# Autodesk Inventor assembly: Aspresor
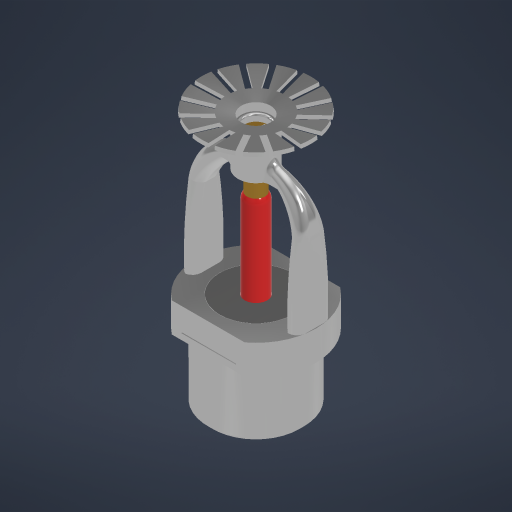
[picture p0: Inventor's stored thumbnail of the model, 512x512]
Saved by Autodesk Inventor 2024 (Build 280153000, 153)
## iProperties
Created: 2024-11-05
Part Number: Aspresor
Document SubType Name: Assembly
Designer: nesto
Author: nesto
## Documents named in this file (3)
- C:\Users\nesto\OneDrive - Universidad de la Sabana\Universidad\2024-2\CAD\Sistema de Riego\Aspresor.iam
- C:\Users\nesto\OneDrive - Universidad de la Sabana\Universidad\2024-2\CAD\Sistema de Riego\parte de abajo.ipt
- C:\Users\nesto\OneDrive - Universidad de la Sabana\Universidad\2024-2\CAD\Sistema de Riego\Parte de arriba aspresor.ipt
## Components (2 placed, 2 different names)
1. parte de abajo:1 — De rotación:1
2. Parte de arriba aspresor:1 — De rotación:1
## Relationships (1: RevoluteJoint 1)
- De rotación:1 [RevoluteJoint]: parte de abajo:1 ↔ Parte de arriba aspresor:1
